# Autodesk Inventor assembly: Pancake_Flexi Pipe Assy
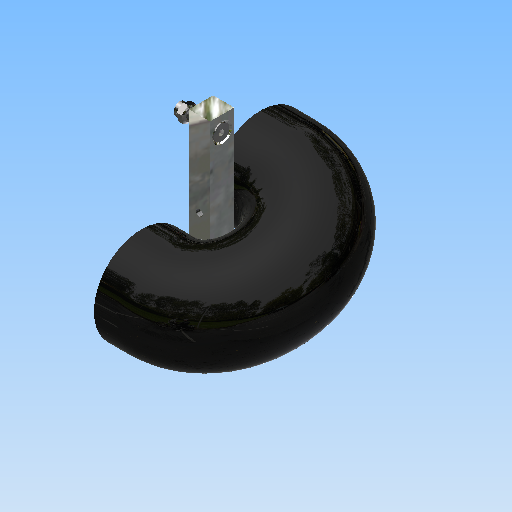
[picture p0: Inventor's stored thumbnail of the model, 512x512]
Saved by Autodesk Inventor 2018.1 (Build 221171000, 171)
## iProperties
Created: 2019-02-26
Part Number: Pancake_Flexi Pipe Assy
Document SubType Name: Assembly
Designer: James
Author: James
## Documents named in this file (6)
- C:\Users\admin\Desktop\Ball-Machine\Pancake Sort\Pancake_Flexi Pipe Assy.iam
- C:\Users\admin\Desktop\Ball-Machine\Pancake Sort\Pancake_Flexi Pipe.ipt
- C:\Users\admin\Desktop\Ball-Machine\Pancake Sort\Pancake_Flexi Pipe Mount.ipt
- C:\Users\admin\Desktop\Ball-Machine\Pancake Sort\Nyloc Nut - M4.ipt
- C:\Users\admin\Desktop\Ball-Machine\Pancake Sort\Socket Csk Screw - (A2) - M4 x  20.ipt
- C:\Users\admin\Desktop\Ball-Machine\Pancake Sort\Socket Csk Screw - (A2) - M4 x  12.ipt
## Components (8 placed, 5 different names)
1. Pancake_Flexi Pipe Mount:1 — Flush:1, Flush:2, Flush:3, Mate:1, Tangent:1, Flush:4, Mate:9, Tangent:2, Mate:10, Mate:12, Mate:13, Tangent:3
2. Pancake_Flexi Pipe:1 — Mate:1, Tangent:1, Flush:4
3. Socket Csk Screw - (A2) - M4 x  12:1
4. Socket Csk Screw - (A2) - M4 x  12:2
5. Nyloc Nut - M4:3 — Mate:10
6. Socket Csk Screw - (A2) - M4 x  20:3 — Mate:9, Tangent:2
7. Nyloc Nut - M4:4 — Mate:13
8. Socket Csk Screw - (A2) - M4 x  20:4 — Mate:12, Tangent:3
## Relationships (18: Mate 9, Flush 6, Tangent 3)
- Flush:1: Pancake_Flexi Pipe Mount:1
- Flush:2: Pancake_Flexi Pipe Mount:1
- Flush:3: Pancake_Flexi Pipe Mount:1
- Mate:1: Pancake_Flexi Pipe Mount:1 ↔ Pancake_Flexi Pipe:1
- Tangent:1: Pancake_Flexi Pipe Mount:1 ↔ Pancake_Flexi Pipe:1
- Flush:4: Pancake_Flexi Pipe Mount:1 ↔ Pancake_Flexi Pipe:1
- [Mate]: Pancake_Flexi Pipe Mount:1 ↔ Socket Csk Screw - (A2) - M4 x  12:1
- [Flush] (-4 mm): Pancake_Flexi Pipe Mount:1 ↔ Socket Csk Screw - (A2) - M4 x  12:1
- [Flush] (-4 mm): Pancake_Flexi Pipe Mount:1 ↔ Socket Csk Screw - (A2) - M4 x  12:2
- [Mate]: Pancake_Flexi Pipe Mount:1 ↔ Socket Csk Screw - (A2) - M4 x  12:2
- [Mate]: Nyloc Nut - M4:3 ↔ Socket Csk Screw - (A2) - M4 x  20:3
- Mate:9: Pancake_Flexi Pipe Mount:1 ↔ Socket Csk Screw - (A2) - M4 x  20:3
- Tangent:2: Pancake_Flexi Pipe Mount:1 ↔ Socket Csk Screw - (A2) - M4 x  20:3
- Mate:10 (5 mm): Pancake_Flexi Pipe Mount:1 ↔ Nyloc Nut - M4:3
- [Mate]: Nyloc Nut - M4:4 ↔ Socket Csk Screw - (A2) - M4 x  20:4
- Mate:12: Pancake_Flexi Pipe Mount:1 ↔ Socket Csk Screw - (A2) - M4 x  20:4
- Mate:13 (5 mm): Pancake_Flexi Pipe Mount:1 ↔ Nyloc Nut - M4:4
- Tangent:3: Pancake_Flexi Pipe Mount:1 ↔ Socket Csk Screw - (A2) - M4 x  20:4
## Named parameters: d14_d11 = 0 mm, d18_d14_d11 = 0 mm
